# Autodesk Inventor assembly: HbSocket
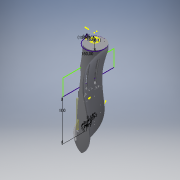
[picture p0: Inventor's stored thumbnail of the model, 180x180]
Saved by Autodesk Inventor 2017 (Build 210142000, 142)
## iProperties
Part Number: HbSocket
Material: 一般
Document SubType Name: Assembly
Designer: sktom
Author: sktom
## Documents named in this file (4)
- D:\OneDrive\CAD\MAJ\hackberry\HACKberry-hardware\3D_69%\Inventor\HbSocketForChild\HbSocket.iam
- D:\OneDrive\CAD\MAJ\hackberry\HACKberry-hardware\3D_69%\Inventor\HbSocketForChild\HbMainFrameA01ForChild.ipt
- D:\OneDrive\CAD\MAJ\hackberry\HACKberry-hardware\3D_69%\Inventor\HbSocketForChild\HbMainFrameB01ForChild.ipt
- D:\OneDrive\CAD\MAJ\hackberry\HACKberry-hardware\3D_69%\Inventor\HbSocketForChild\HbBatteryCase01.ipt
## Components (3 placed, 3 different names)
1. HbMainFrameA01ForChild:1 — 挿入:1, 挿入:2
2. HbMainFrameB01ForChild:1 — 挿入:1, 挿入:2, 挿入:3, 挿入:4, フラッシュ:1
3. HbBatteryCase01:2 — 挿入:3, 挿入:4, フラッシュ:1
## Relationships (5: Insert 4, Flush 1)
- 挿入:1 [Insert]: HbMainFrameA01ForChild:1 ↔ HbMainFrameB01ForChild:1
- 挿入:2 [Insert]: HbMainFrameA01ForChild:1 ↔ HbMainFrameB01ForChild:1
- 挿入:3 [Insert]: HbMainFrameB01ForChild:1 ↔ HbBatteryCase01:2
- 挿入:4 [Insert]: HbMainFrameB01ForChild:1 ↔ HbBatteryCase01:2
- フラッシュ:1 [Flush]: HbMainFrameB01ForChild:1 ↔ HbBatteryCase01:2
